# Autodesk Inventor assembly: Double Acting Piston_MIR
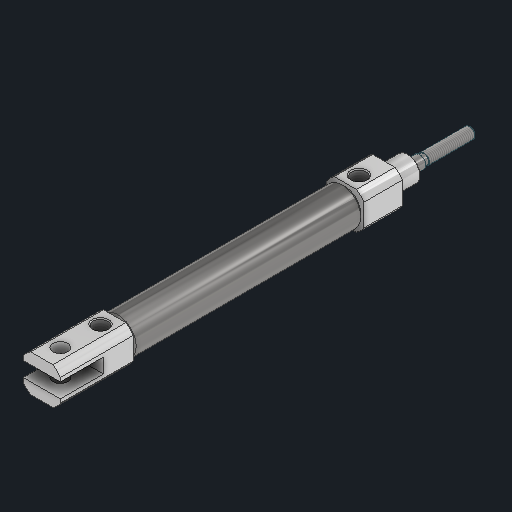
[picture p0: Inventor's stored thumbnail of the model, 512x512]
Saved by Autodesk Inventor 2024 (Build 280153000, 153)
## iProperties
Created: 2022-09-23
Part Number: Double Acting Piston_MIR
Document SubType Name: Assembly
Designer: Averey Ku
Mass: 9.29214 g
Surface Area: 91.0706 cm^2
Volume: 9.29214 cm^3
Density: 1 g/cm^3
Author: maxxw
## Documents named in this file (3)
- D:\vex_robotics\hardware\cad\zoomba_v0.3\arm\Double Acting Piston_MIR.iam
- D:\vex_robotics\hardware\cad\zoomba_v0.3\arm\Double Acting Piston Body_MIR.ipt
- D:\vex_robotics\hardware\cad\zoomba_v0.3\arm\Double Acting Piston Rod_MIR.ipt
## Components (2 placed, 2 different names)
1. Double Acting Piston Body_MIR:1 — Mate:2, Mate:1
2. Double Acting Piston Rod_MIR:1 — Mate:2, Mate:1
## Relationships (2: Mate 2)
- Mate:2: Double Acting Piston Body_MIR:1 ↔ Double Acting Piston Rod_MIR:1
- Mate:1: Double Acting Piston Body_MIR:1 ↔ Double Acting Piston Rod_MIR:1
